# Autodesk Inventor assembly: Ensamble_Áng_Desb
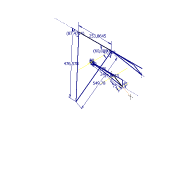
[picture p0: Inventor's stored thumbnail of the model, 180x180]
Saved by Autodesk Inventor 2021 (Build 250183000, 183)
## iProperties
Created: 2021-06-14
Part Number: Ensamble_Áng_Desb
Document SubType Name: Assembly
Designer: Santiago
Author: Santiago
## Documents named in this file (5)
- C:\Users\user\Desktop\Ingeniería Mecánica UN\6. Sexto Semestre\Mecanismos\Archivos_AC3_Marín_Becerra\Ensamble_Áng_Desb.iam
- C:\Users\user\Desktop\Ingeniería Mecánica UN\6. Sexto Semestre\Mecanismos\Archivos_AC3_Marín_Becerra\Acoplador.ipt
- C:\Users\user\Desktop\Ingeniería Mecánica UN\6. Sexto Semestre\Mecanismos\Archivos_AC3_Marín_Becerra\Bancada.ipt
- C:\Users\user\Desktop\Ingeniería Mecánica UN\6. Sexto Semestre\Mecanismos\Archivos_AC3_Marín_Becerra\Corredera.ipt
- C:\Users\user\Desktop\Ingeniería Mecánica UN\6. Sexto Semestre\Mecanismos\Archivos_AC3_Marín_Becerra\Manivela.ipt
## Components (4 placed, 4 different names)
1. Acoplador:1 — Mate:3, Mate:4, Mate:5, Mate:6
2. Bancada:1 — Mate:1, Mate:2, Mate:7, Angle:1
3. Corredera:1 — Mate:5, Mate:6, Mate:7
4. Manivela:1 — Mate:1, Mate:2, Mate:3, Mate:4, Angle:1
## Relationships (8: Mate 7, Angle 1)
- Mate:1: Bancada:1 ↔ Manivela:1
- Mate:2: Bancada:1 ↔ Manivela:1
- Mate:3: Acoplador:1 ↔ Manivela:1
- Mate:4: Acoplador:1 ↔ Manivela:1
- Mate:5: Acoplador:1 ↔ Corredera:1
- Mate:6: Acoplador:1 ↔ Corredera:1
- Mate:7: Bancada:1 ↔ Corredera:1
- Angle:1 (150 deg): Bancada:1 ↔ Manivela:1
